# Autodesk Inventor assembly: SELF-LUBRIFICATING ROD END
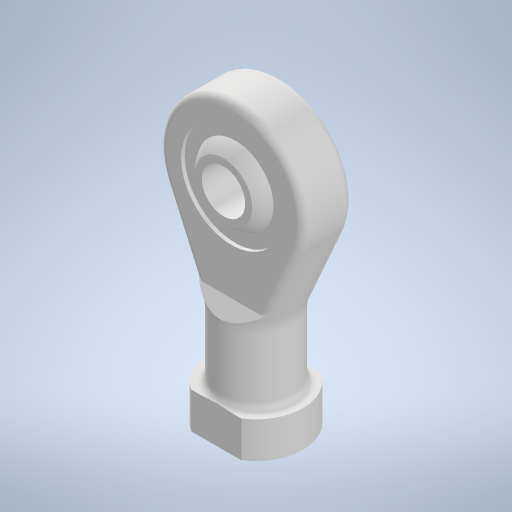
[picture p0: Inventor's stored thumbnail of the model, 512x512]
Saved by Autodesk Inventor 2023 (Build 270158000, 158)
## iProperties
Created: 2023-02-24
Part Number: SELF-LUBRIFICATING ROD END
Document SubType Name: Assembly
Designer: roota
Author: roota
## Documents named in this file (3)
- D:\GitHub\NTUST-Mechanical-Design\Ball stabilization mechanism\3D CAD files\Mechanical Part CAD files\Hardware Parts\SELF-LUBRIFICATING ROD END\SELF-LUBRIFICATING ROD END.iam
- D:\GitHub\NTUST-Mechanical-Design\Ball stabilization mechanism\3D CAD files\Mechanical Part CAD files\Hardware Parts\SELF-LUBRIFICATING ROD END\Ball_6mm.ipt
- D:\GitHub\NTUST-Mechanical-Design\Ball stabilization mechanism\3D CAD files\Mechanical Part CAD files\Hardware Parts\SELF-LUBRIFICATING ROD END\End_6mm.ipt
## Components (2 placed, 2 different names)
1. Ball_6mm:1 — Mate:1
2. End_6mm:1 — Mate:1
## Relationships (1: Mate 1)
- Mate:1: Ball_6mm:1 ↔ End_6mm:1
